# Autodesk Inventor assembly: Сборка
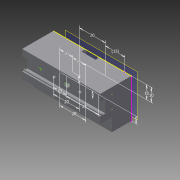
[picture p0: Inventor's stored thumbnail of the model, 180x180]
Saved by Autodesk Inventor 2015 (Build 190159000, 159)
## iProperties
Created: 2016-04-08
Part Number: Сборка
Document SubType Name: Assembly
Designer: Andreas
Author: Andreas
## Documents named in this file (3)
- C:\Users\Andreas\Documents\GitHub\LaserProject\ласт_ворк_v1.5.3\каретка+деталь к ней\Detal+Karetka.iam
- C:\Users\Andreas\Documents\GitHub\LaserProject\ласт_ворк_v1.5.3\каретка+деталь к ней\Karetka.ipt
- C:\Users\Andreas\Documents\GitHub\LaserProject\ласт_ворк_v1.5.3\каретка+деталь к ней\DetalKKaretke.ipt
## Components (2 placed, 2 different names)
1. Karetka:1 — Rigid:1
2. DetalKKaretke:1 — Rigid:1
## Relationships (1: WeldJoint 1)
- Rigid:1 [WeldJoint]: Karetka:1 ↔ DetalKKaretke:1
